# Autodesk Inventor assembly: cRIO-FRC
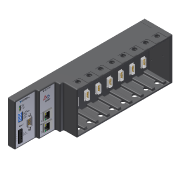
[picture p0: Inventor's stored thumbnail of the model, 180x180]
Saved by Autodesk Inventor 2011 (Build 150239000, 239)
## iProperties
Category: FIRST
Manager: Ed Sparks
Company: FirstCadLibrary
Shininess: 64.0
Length Units: 11272
Angle Units: 11279
Time Units: 11290
Mass Units: 11286
Length Display Precision: 3
Angle Display Precision: 2
Compacted: True
Part Number: cRIO-FRC
Document SubType Name: Assembly
Created: 2008-12-10
Designer: Ed Sparks
Project: FIRST
Catalog Web Link: www.firstcadlibrary.com
Engineer: Ed Sparks
Density: 0.0
Volumn: 0.0
Area: 0.0
PropertySet Name: Model Information
Control State: 0
Master: False
Checked Out: False
Author: Ed Sparks
Keywords: FIRST
## Documents named in this file (6)
- R:\2010-2011\CMO\Web Site\CADalog\Electonics\cRIO 1764\cRIO-FRC 1764.iam
- R:\2010-2011\CMO\Web Site\CADalog\Electonics\cRIO 1764\cRIO Pad 1764.ipt
- R:\2010-2011\CMO\Web Site\CADalog\Electonics\cRIO 1764\BackPlate 1764.ipt
- R:\2010-2011\CMO\Web Site\CADalog\Electonics\cRIO 1764\cRIO Chassis 1764.ipt
- R:\2010-2011\CMO\Web Site\CADalog\Electonics\cRIO 1764\cRIO Screws 1764.ipt
- R:\2010-2011\CMO\Web Site\CADalog\Electonics\cRIO 1764\cRIO PCB 1764.iam
## Components (12 placed, 5 different names)
1. cRIO-FRC Chassis:1 — Mate:1, Mate:2, Mate:3, Mate:4, Mate:5, Mate:6, Mate:7, Mate:8
2. BackPlate 1764:1 — Mate:1, Mate:2, Insert:1, Insert:2, Insert:3, Insert:4, Insert:5, Insert:6, Insert:7, Insert:8
3. cRIO Pad 1764:1 — Mate:3, Mate:4, Mate:5
4. cRIO PCB 1764:1 [sub-assembly] — Mate:6, Mate:7, Mate:8
5. cRIO Screws 1764:1 — Insert:1
6. cRIO Screws 1764:2 — Insert:2
7. cRIO Screws 1764:3 — Insert:3
8. cRIO Screws 1764:4 — Insert:4
9. cRIO Screws 1764:5 — Insert:5
10. cRIO Screws 1764:6 — Insert:6
11. cRIO Screws 1764:7 — Insert:7
12. cRIO Screws 1764:8 — Insert:8
## Relationships (16: Mate 8, Insert 8)
- Mate:1: cRIO-FRC Chassis:1 ↔ BackPlate 1764:1
- Mate:2: cRIO-FRC Chassis:1 ↔ BackPlate 1764:1
- Mate:3: cRIO-FRC Chassis:1 ↔ cRIO Pad 1764:1
- Mate:4 (5.08 mm): cRIO-FRC Chassis:1 ↔ cRIO Pad 1764:1
- Mate:5 (3.81 mm): cRIO-FRC Chassis:1 ↔ cRIO Pad 1764:1
- Mate:6: cRIO-FRC Chassis:1 ↔ cRIO PCB 1764:1
- Mate:7: cRIO-FRC Chassis:1 ↔ cRIO PCB 1764:1
- Mate:8: cRIO-FRC Chassis:1 ↔ cRIO PCB 1764:1
- Insert:1: BackPlate 1764:1 ↔ cRIO Screws 1764:1
- Insert:2: BackPlate 1764:1 ↔ cRIO Screws 1764:2
- Insert:3: BackPlate 1764:1 ↔ cRIO Screws 1764:3
- Insert:4: BackPlate 1764:1 ↔ cRIO Screws 1764:4
- Insert:5: BackPlate 1764:1 ↔ cRIO Screws 1764:5
- Insert:6: BackPlate 1764:1 ↔ cRIO Screws 1764:6
- Insert:7: BackPlate 1764:1 ↔ cRIO Screws 1764:7
- Insert:8: BackPlate 1764:1 ↔ cRIO Screws 1764:8
